# Autodesk Inventor assembly: Assembly
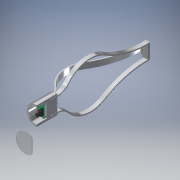
[picture p0: Inventor's stored thumbnail of the model, 180x180]
Saved by Autodesk Inventor 2016 (Build 200138000, 138)
## iProperties
Created: 2016-06-15
Part Number: Assembly
Document SubType Name: Assembly
Designer: Andres
Author: Andres
## Documents named in this file (8)
- Z:\Documents\repositorios\BoreholeCamera\CAD_Probe\Assembly\Assembly.iam
- Z:\Documents\repositorios\BoreholeCamera\CAD_Probe\Enclosure\Parts\Enclosure.ipt
- Z:\Documents\repositorios\BoreholeCamera\CAD_Probe\Camera\Assembly\Assembly.iam
- Z:\Documents\repositorios\BoreholeCamera\CAD_Probe\Enclosure\Parts\Cover.ipt
- Z:\Documents\repositorios\BoreholeCamera\CAD_Probe\Enclosure\Parts\8inch_Fin.ipt
- Z:\Documents\repositorios\BoreholeCamera\CAD_Probe\Enclosure\Parts\Bottom.ipt
- Z:\Documents\repositorios\BoreholeCamera\CAD_Probe\Enclosure\Parts\STEP\91075A212_18-8 SS MALE-FEM THRDED HEX STANDOFF.ipt
- Z:\Documents\repositorios\BoreholeCamera\CAD_Probe\Enclosure\Parts\90910A680_LOW-PROFILE BUTTON HEAD TORX MACHINE SCREW.ipt
## Components (16 placed, 7 different names)
1. Enclosure:1 — Mate:1, Mate:2, Insert:1, Insert:2, Rigid:7
2. Cover:1
3. 8inch_Fin:1
4. 8inch_Fin:2
5. 8inch_Fin:3 — Rigid:6
6. 8inch_Fin:4
7. Bottom:1 — Rigid:6
8. 91075A212_18-8 SS MALE-FEM THRDED HEX STANDOFF:3 — Mate:1
9. 91075A212_18-8 SS MALE-FEM THRDED HEX STANDOFF:4 — Mate:2
10. 91075A212_18-8 SS MALE-FEM THRDED HEX STANDOFF:5 — Insert:1
11. 91075A212_18-8 SS MALE-FEM THRDED HEX STANDOFF:6 — Insert:2
12. Assembly:1 [sub-assembly] — Rigid:7, Rotational:1, Rotational:2, Rotational:3, Rotational:4
13. 90910A680_LOW-PROFILE BUTTON HEAD TORX MACHINE SCREW:1 — Rotational:1
14. 90910A680_LOW-PROFILE BUTTON HEAD TORX MACHINE SCREW:2 — Rotational:2
15. 90910A680_LOW-PROFILE BUTTON HEAD TORX MACHINE SCREW:3 — Rotational:3
16. 90910A680_LOW-PROFILE BUTTON HEAD TORX MACHINE SCREW:4 — Rotational:4
## Relationships (10: RevoluteJoint 4, WeldJoint 2, Mate 2, Insert 2)
- Rigid:6 [WeldJoint]: 8inch_Fin:3 ↔ Bottom:1
- Mate:1: Enclosure:1 ↔ 91075A212_18-8 SS MALE-FEM THRDED HEX STANDOFF:3
- Mate:2: Enclosure:1 ↔ 91075A212_18-8 SS MALE-FEM THRDED HEX STANDOFF:4
- Insert:1: Enclosure:1 ↔ 91075A212_18-8 SS MALE-FEM THRDED HEX STANDOFF:5
- Insert:2: Enclosure:1 ↔ 91075A212_18-8 SS MALE-FEM THRDED HEX STANDOFF:6
- Rigid:7 [WeldJoint] (9.525 mm): Enclosure:1 ↔ Assembly:1
- Rotational:1 [RevoluteJoint]: Assembly:1 ↔ 90910A680_LOW-PROFILE BUTTON HEAD TORX MACHINE SCREW:1
- Rotational:2 [RevoluteJoint]: Assembly:1 ↔ 90910A680_LOW-PROFILE BUTTON HEAD TORX MACHINE SCREW:2
- Rotational:3 [RevoluteJoint]: Assembly:1 ↔ 90910A680_LOW-PROFILE BUTTON HEAD TORX MACHINE SCREW:3
- Rotational:4 [RevoluteJoint]: Assembly:1 ↔ 90910A680_LOW-PROFILE BUTTON HEAD TORX MACHINE SCREW:4
